# Autodesk Inventor assembly: corners 20feet
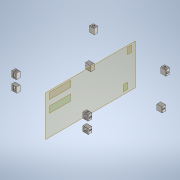
[picture p0: Inventor's stored thumbnail of the model, 180x180]
Saved by Autodesk Inventor 2020 (Build 240168000, 168)
## iProperties
Created: 2022-11-18
Part Number: corners 20feet
Document SubType Name: Assembly
Designer: super
Author: super
## Documents named in this file (3)
- C:\desk\promissionsave\inventor\container\corners 20feet.iam
- C:\desk\promissionsave\inventor\container\corners bottom.iam
- C:\desk\promissionsave\inventor\container\corners top.iam
## Components (4 placed, 2 different names)
1. corners bottom:1 [sub-assembly] — Flush:1, Mate:1, Flush:2, Flush:3, Flush:4, Flush:5, Mate:2
2. corners bottom:2 [sub-assembly] — Mate:1, Flush:2, Flush:3
3. corners top:1 [sub-assembly] — Flush:4, Flush:5, Mate:2
4. corners top:2 [sub-assembly]
## Relationships (7: Flush 5, Mate 2)
- Flush:1: corners bottom:1
- Mate:1 (200 mm): corners bottom:1 ↔ corners bottom:2
- Flush:2: corners bottom:1 ↔ corners bottom:2
- Flush:3: corners bottom:1 ↔ corners bottom:2
- Flush:4: corners bottom:1 ↔ corners top:1
- Flush:5: corners bottom:1 ↔ corners top:1
- Mate:2 (2354.8 mm): corners bottom:1 ↔ corners top:1
